# Autodesk Inventor assembly: ParticleLauncherwCollector
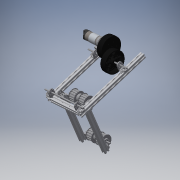
[picture p0: Inventor's stored thumbnail of the model, 180x180]
Saved by Autodesk Inventor 2016 (Build 200138000, 138)
## iProperties
Created: 2016-10-12
Part Number: ParticleLauncherwCollector
Document SubType Name: Assembly
Designer: Delta
Author: Delta
## Documents named in this file (13)
- C:\Robotics\CAD\2016-17_CAD\ParticleLauncherwCollector.iam
- C:\Robotics\CAD\COTSParts\Actobotics\555 parts\555116.ipt
- C:\Robotics\CAD\COTSParts\Actobotics\am-3102NeveRest20 (1).ipt
- C:\Robotics\CAD\COTSParts\Actobotics\634 parts\634088.ipt
- C:\Robotics\CAD\COTSParts\Wheels\4in Wheel Intergreated Hub 8mm Rev2.ipt
- C:\Robotics\CAD\COTSParts\Bearings - AndyMark\Bearing 250 ID 500 OD flanged.ipt
- C:\Robotics\CAD\COTSParts\Actobotics\545 parts\545400.ipt
- C:\Robotics\CAD\COTSParts\Bosch Extrusion\6mm block nut M4.ipt
- C:\Robotics\CAD\COTSParts\Actobotics\585 parts\585494.ipt
- C:\Robotics\CAD\COTSParts\Bosch Extrusion\Bosch 20x20 - 7.184 Part.Shoot.ipt
- C:\Robotics\CAD\COTSParts\Bosch Extrusion\Gusset 20x20 w screws.ipt
- C:\Robotics\CAD\2016-17_CAD\BoschCollector.iam
- C:\Robotics\CAD\COTSParts\Bosch Extrusion\Bosch 20x20 13 in.ipt
## Components (33 placed, 12 different names)
1. 555116:1 — Insert:15, Insert:35, Insert:36
2. am-3102NeveRest20 (1):1 — Insert:15, Insert:34
3. 634088:1 — Insert:17, Insert:42, Insert:57
4. 4in Wheel Intergreated Hub 8mm Rev2:1 — Insert:17
5. 4in Wheel Intergreated Hub 8mm Rev2:2 — Insert:34
6. Bearing 250 ID 500 OD flanged:2 — Insert:41, Insert:42
7. Bearing 250 ID 500 OD flanged:3 — Insert:48, Insert:57
8. 545400:1 — Insert:45, Insert:46, Insert:48, Mate:38
9. 545400:2 — Insert:39, Insert:40, Insert:41, Mate:41
10. 6mm block nut M4:1 — Insert:44, Mate:51
11. 6mm block nut M4:2 — Insert:43, Mate:49, Mate:50
12. 6mm block nut M4:4 — Insert:45
13. 6mm block nut M4:5 — Insert:46
14. 6mm block nut M4:6 — Insert:39
15. 6mm block nut M4:7 — Insert:40, Mate:46, Mate:47
16. 585494:2 — Insert:35, Insert:36, Insert:43, Insert:44, Mate:38
17. 6mm block nut M4:8 — Insert:60
18. 6mm block nut M4:9 — Insert:58, Mate:44
19. 6mm block nut M4:10 — Flush:1, Insert:59, Mate:42, Flush:2, Mate:43
20. 6mm block nut M4:11 — Insert:61
21. 634088:2
22. 545400:3 — Insert:55, Insert:58, Insert:59
23. 545400:4 — Insert:56, Insert:60, Insert:61
24. Bearing 250 ID 500 OD flanged:4 — Insert:56
25. Bearing 250 ID 500 OD flanged:5 — Insert:55
26. Bosch 20x20 - 7.184 Part.Shoot:1 — Mate:30, Mate:31, Mate:34, Mate:35, Mate:45, Flush:3, Flush:4, Flush:5, Flush:6, Mate:48
27. Gusset 20x20 w screws:1 — Mate:30, Mate:31, Mate:53
28. Gusset 20x20 w screws:2 — Mate:34, Mate:35, Mate:52
29. BoschCollector:1 [sub-assembly] — Mate:41, Mate:60, Mate:61, Mate:62, Mate:63
30. Bosch 20x20 13 in:1 — Flush:5, Flush:6, Mate:48, Mate:49, Mate:50, Mate:51, Mate:53, Mate:63
31. Bosch 20x20 13 in:2 — Flush:1, Mate:42, Flush:2, Mate:43, Mate:44, Mate:45, Flush:3, Flush:4, Mate:46, Mate:47, Mate:52, Mate:59
32. Gusset 20x20 w screws:3 — Mate:62
33. Gusset 20x20 w screws:4 — Mate:59, Mate:60, Mate:61
## Relationships (50: Mate 23, Insert 21, Flush 6)
- Insert:15 (-9.525 mm): 555116:1 ↔ am-3102NeveRest20 (1):1
- Insert:17 (63.5 mm): 634088:1 ↔ 4in Wheel Intergreated Hub 8mm Rev2:1
- Insert:34 (-10.16 mm): am-3102NeveRest20 (1):1 ↔ 4in Wheel Intergreated Hub 8mm Rev2:2
- Insert:35: 555116:1 ↔ 585494:2
- Insert:36: 555116:1 ↔ 585494:2
- Insert:39: 545400:2 ↔ 6mm block nut M4:6
- Insert:40: 545400:2 ↔ 6mm block nut M4:7
- Insert:41: Bearing 250 ID 500 OD flanged:2 ↔ 545400:2
- Insert:42 (41.2369 mm): 634088:1 ↔ Bearing 250 ID 500 OD flanged:2
- Insert:43: 6mm block nut M4:2 ↔ 585494:2
- Insert:44: 6mm block nut M4:1 ↔ 585494:2
- Insert:45: 545400:1 ↔ 6mm block nut M4:4
- Insert:46: 545400:1 ↔ 6mm block nut M4:5
- Insert:48: Bearing 250 ID 500 OD flanged:3 ↔ 545400:1
- Insert:55: 545400:3 ↔ Bearing 250 ID 500 OD flanged:5
- Insert:56: 545400:4 ↔ Bearing 250 ID 500 OD flanged:4
- Insert:57 (41.2369 mm): 634088:1 ↔ Bearing 250 ID 500 OD flanged:3
- Mate:30: Bosch 20x20 - 7.184 Part.Shoot:1 ↔ Gusset 20x20 w screws:1
- Mate:31: Bosch 20x20 - 7.184 Part.Shoot:1 ↔ Gusset 20x20 w screws:1
- Mate:34: Bosch 20x20 - 7.184 Part.Shoot:1 ↔ Gusset 20x20 w screws:2
- Mate:35: Bosch 20x20 - 7.184 Part.Shoot:1 ↔ Gusset 20x20 w screws:2
- Mate:38 (7.62 mm): 545400:1 ↔ 585494:2
- Mate:41 (162.5854 mm): 545400:2 ↔ BoschCollector:1
- Flush:1: 6mm block nut M4:10 ↔ Bosch 20x20 13 in:2
- Insert:58: 6mm block nut M4:9 ↔ 545400:3
- Insert:59: 6mm block nut M4:10 ↔ 545400:3
- Insert:60: 6mm block nut M4:8 ↔ 545400:4
- Insert:61: 6mm block nut M4:11 ↔ 545400:4
- Mate:42: 6mm block nut M4:10 ↔ Bosch 20x20 13 in:2
- Flush:2: 6mm block nut M4:10 ↔ Bosch 20x20 13 in:2
- Mate:43: 6mm block nut M4:10 ↔ Bosch 20x20 13 in:2
- Mate:44: 6mm block nut M4:9 ↔ Bosch 20x20 13 in:2
- Mate:45: Bosch 20x20 - 7.184 Part.Shoot:1 ↔ Bosch 20x20 13 in:2
- Flush:3: Bosch 20x20 - 7.184 Part.Shoot:1 ↔ Bosch 20x20 13 in:2
- Flush:4: Bosch 20x20 - 7.184 Part.Shoot:1 ↔ Bosch 20x20 13 in:2
- Mate:46: 6mm block nut M4:7 ↔ Bosch 20x20 13 in:2
- Mate:47: 6mm block nut M4:7 ↔ Bosch 20x20 13 in:2
- Flush:5: Bosch 20x20 - 7.184 Part.Shoot:1 ↔ Bosch 20x20 13 in:1
- Flush:6: Bosch 20x20 - 7.184 Part.Shoot:1 ↔ Bosch 20x20 13 in:1
- Mate:48: Bosch 20x20 - 7.184 Part.Shoot:1 ↔ Bosch 20x20 13 in:1
- Mate:49: 6mm block nut M4:2 ↔ Bosch 20x20 13 in:1
- Mate:50: 6mm block nut M4:2 ↔ Bosch 20x20 13 in:1
- Mate:51: 6mm block nut M4:1 ↔ Bosch 20x20 13 in:1
- Mate:52: Gusset 20x20 w screws:2 ↔ Bosch 20x20 13 in:2
- Mate:53: Gusset 20x20 w screws:1 ↔ Bosch 20x20 13 in:1
- Mate:59: Bosch 20x20 13 in:2 ↔ Gusset 20x20 w screws:4
- Mate:60: BoschCollector:1 ↔ Gusset 20x20 w screws:4
- Mate:61: BoschCollector:1 ↔ Gusset 20x20 w screws:4
- Mate:62: BoschCollector:1 ↔ Gusset 20x20 w screws:3
- Mate:63: BoschCollector:1 ↔ Bosch 20x20 13 in:1
